# Autodesk Inventor assembly: Sharpie-Fine-Point
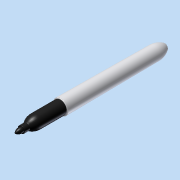
[picture p0: Inventor's stored thumbnail of the model, 180x180]
Saved by Autodesk Inventor 2012 (Build 160160000, 160)
## iProperties
Created: 2015-03-22
Part Number: Sharpie-Fine-Point
Document SubType Name: Assembly
Designer: Jason
Author: Jason
## Documents named in this file (6)
- C:\Users\Jason\Documents\Dropbox\Synio\Synio Spray Pen\Product Design\CAD\Markers\Sharpie Fine Point\Sharpie-Fine-Point.iam
- C:\Users\Jason\Documents\Dropbox\Synio\Synio Spray Pen\Product Design\CAD\Markers\Sharpie Fine Point\Body.ipt
- C:\Users\Jason\Documents\Dropbox\Synio\Synio Spray Pen\Product Design\CAD\Markers\Sharpie Fine Point\Body_Sleeve.ipt
- C:\Users\Jason\Documents\Dropbox\Synio\Synio Spray Pen\Product Design\CAD\Markers\Sharpie Fine Point\Nib.ipt
- C:\Users\Jason\Documents\Dropbox\Synio\Synio Spray Pen\Product Design\CAD\Markers\Sharpie Fine Point\Cartridge.iam
- C:\Users\Jason\Documents\Dropbox\Synio\Synio Spray Pen\Product Design\CAD\Markers\Sharpie Fine Point\Cap.ipt
## Components (5 placed, 5 different names)
1. Body:1 — Insert:1, Mate:3, Flush:1, Mate:4, Mate:5, Mate:6
2. Body_Sleeve:1 — Insert:1, Mate:1, Mate:2, Mate:4
3. Nib:1 — Mate:1, Mate:2, Mate:3
4. Cartridge:1 [sub-assembly] — Mate:5, Mate:6
5. Cap:1 — Flush:2, Mate:7
## Relationships (10: Mate 7, Flush 2, Insert 1)
- Insert:1: Body:1 ↔ Body_Sleeve:1
- Mate:1: Body_Sleeve:1 ↔ Nib:1
- Mate:2 (-5.5 mm): Body_Sleeve:1 ↔ Nib:1
- Mate:3: Body:1 ↔ Nib:1
- Flush:1: Body:1
- Mate:4: Body:1 ↔ Body_Sleeve:1
- Mate:5: Body:1 ↔ Cartridge:1
- Mate:6: Body:1 ↔ Cartridge:1
- Flush:2: Cap:1
- Mate:7: Cap:1
